# Autodesk Inventor assembly: 165565807 18793263 170831 DFM-12-100-P-A-GF---(fdt_d_0)
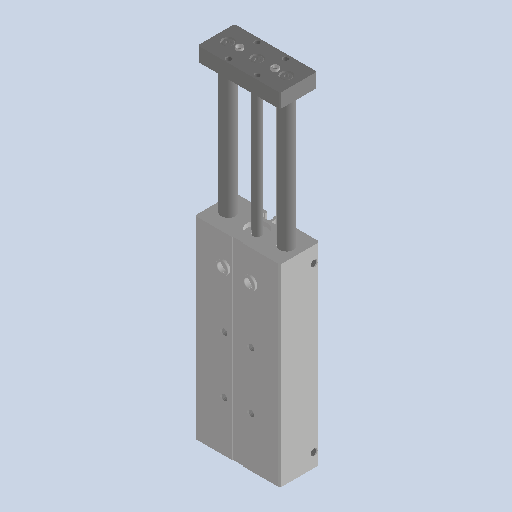
[picture p0: Inventor's stored thumbnail of the model, 512x512]
Saved by Autodesk Inventor 2025.1 (Build 291241000, 241)
## iProperties
Category: PARTsolutions
Created: 2025-06-15
Part Number: 165565807 18793263 170831 DFM-12-100-P-A-GF---(fdt_d_0)
Catalog Web Link: www.cadenas.de
Description: -
Document SubType Name: Assembly
Designer: psAdmin
Mass: 229.263 g
Surface Area: 644.764 cm^2
Volume: 221.571 cm^3
Density: 1.03471 g/cm^3
CREATOR: CADENAS GmbH
Author: Cadenas PARTsolutions
## Documents named in this file (5)
- C:\Users\Erik\Erik\Hochschule\3. Semester\CAD\CAD-Paspa\Useless Box\Kaufteile\Festo_Fuehrungszylinder_100\165565807 18793263 170831 DFM-12-100-P-A-GF---(fdt_d_0).iam
- C:\Users\Erik\Erik\Hochschule\3. Semester\CAD\CAD-Paspa\Useless Box\Kaufteile\Festo_Fuehrungszylinder_100\170831 DFM-12-100-P-A-GF---(Z).ipt
- C:\Users\Erik\Erik\Hochschule\3. Semester\CAD\CAD-Paspa\Useless Box\Kaufteile\Festo_Fuehrungszylinder_100\170831 DFM-12-100-P-A-GF---(K).ipt
- C:\Users\Erik\Erik\Hochschule\3. Semester\CAD\CAD-Paspa\Useless Box\Kaufteile\Festo_Fuehrungszylinder_100\8146543 ZBH-5-B.ipt
- C:\Users\Erik\Erik\Hochschule\3. Semester\CAD\CAD-Paspa\Useless Box\Kaufteile\Festo_Fuehrungszylinder_100\8137184 ZBH-9-B.ipt
## Components (8 placed, 4 different names)
1. 170831 DFM-12-100-P-A-GF---(Z):1 — dfm_z_XY@1 <-> dfm_k_XY@2, dfm_z_Z@1 <-> dfm_k_Z@2, dfm_z_YZ@1 <-> dfm_k_YZ@2, HUELSE2_1_XY@1 <-> insert_XY@5, HUELSE2_1_Z@1 <-> insert_Z@5, HUELSE2_1_YZ@1 <-> insert_YZ@5, HUELSE2_2_XY@1 <-> insert_XY@6, HUELSE2_2_Z@1 <-> insert_Z@6, HUELSE2_2_YZ@1 <-> insert_YZ@6, HUELSE1_1_XY@1 <-> insert_XY@7, HUELSE1_1_Z@1 <-> insert_Z@7, HUELSE1_1_YZ@1 <-> insert_YZ@7, HUELSE1_2_XY@1 <-> insert_XY@8, HUELSE1_2_Z@1 <-> insert_Z@8, HUELSE1_2_YZ@1 <-> insert_YZ@8
2. 170831 DFM-12-100-P-A-GF---(K):1 — dfm_z_XY@1 <-> dfm_k_XY@2, dfm_z_Z@1 <-> dfm_k_Z@2, dfm_z_YZ@1 <-> dfm_k_YZ@2, HUELSE3_1_XY@2 <-> insert_XY@3, HUELSE3_1_Z@2 <-> insert_Z@3, HUELSE3_1_YZ@2 <-> insert_YZ@3, HUELSE3_2_XY@2 <-> insert_XY@4, HUELSE3_2_Z@2 <-> insert_Z@4, HUELSE3_2_YZ@2 <-> insert_YZ@4
3. 8146543 ZBH-5-B:1 — HUELSE3_1_XY@2 <-> insert_XY@3, HUELSE3_1_Z@2 <-> insert_Z@3, HUELSE3_1_YZ@2 <-> insert_YZ@3
4. 8146543 ZBH-5-B:2 — HUELSE3_2_XY@2 <-> insert_XY@4, HUELSE3_2_Z@2 <-> insert_Z@4, HUELSE3_2_YZ@2 <-> insert_YZ@4
5. 8137184 ZBH-9-B:1 — HUELSE2_1_XY@1 <-> insert_XY@5, HUELSE2_1_Z@1 <-> insert_Z@5, HUELSE2_1_YZ@1 <-> insert_YZ@5
6. 8137184 ZBH-9-B:2 — HUELSE2_2_XY@1 <-> insert_XY@6, HUELSE2_2_Z@1 <-> insert_Z@6, HUELSE2_2_YZ@1 <-> insert_YZ@6
7. 8146543 ZBH-5-B:3 — HUELSE1_1_XY@1 <-> insert_XY@7, HUELSE1_1_Z@1 <-> insert_Z@7, HUELSE1_1_YZ@1 <-> insert_YZ@7
8. 8146543 ZBH-5-B:4 — HUELSE1_2_XY@1 <-> insert_XY@8, HUELSE1_2_Z@1 <-> insert_Z@8, HUELSE1_2_YZ@1 <-> insert_YZ@8
## Relationships (21: Mate 12, Angle 7, Flush 2)
- dfm_z_XY@1 <-> dfm_k_XY@2 [Mate]: 170831 DFM-12-100-P-A-GF---(Z):1 ↔ 170831 DFM-12-100-P-A-GF---(K):1
- dfm_z_Z@1 <-> dfm_k_Z@2 [Mate]: 170831 DFM-12-100-P-A-GF---(Z):1 ↔ 170831 DFM-12-100-P-A-GF---(K):1
- dfm_z_YZ@1 <-> dfm_k_YZ@2 [Angle] (0 deg): 170831 DFM-12-100-P-A-GF---(Z):1 ↔ 170831 DFM-12-100-P-A-GF---(K):1
- HUELSE3_1_XY@2 <-> insert_XY@3 [Flush]: 170831 DFM-12-100-P-A-GF---(K):1 ↔ 8146543 ZBH-5-B:1
- HUELSE3_1_Z@2 <-> insert_Z@3 [Mate]: 170831 DFM-12-100-P-A-GF---(K):1 ↔ 8146543 ZBH-5-B:1
- HUELSE3_1_YZ@2 <-> insert_YZ@3 [Angle] (0 deg): 170831 DFM-12-100-P-A-GF---(K):1 ↔ 8146543 ZBH-5-B:1
- HUELSE3_2_XY@2 <-> insert_XY@4 [Flush]: 170831 DFM-12-100-P-A-GF---(K):1 ↔ 8146543 ZBH-5-B:2
- HUELSE3_2_Z@2 <-> insert_Z@4 [Mate]: 170831 DFM-12-100-P-A-GF---(K):1 ↔ 8146543 ZBH-5-B:2
- HUELSE3_2_YZ@2 <-> insert_YZ@4 [Angle] (0 deg): 170831 DFM-12-100-P-A-GF---(K):1 ↔ 8146543 ZBH-5-B:2
- HUELSE2_1_XY@1 <-> insert_XY@5 [Mate]: 170831 DFM-12-100-P-A-GF---(Z):1 ↔ 8137184 ZBH-9-B:1
- HUELSE2_1_Z@1 <-> insert_Z@5 [Mate]: 170831 DFM-12-100-P-A-GF---(Z):1 ↔ 8137184 ZBH-9-B:1
- HUELSE2_1_YZ@1 <-> insert_YZ@5 [Angle] (0 deg): 170831 DFM-12-100-P-A-GF---(Z):1 ↔ 8137184 ZBH-9-B:1
- HUELSE2_2_XY@1 <-> insert_XY@6 [Mate]: 170831 DFM-12-100-P-A-GF---(Z):1 ↔ 8137184 ZBH-9-B:2
- HUELSE2_2_Z@1 <-> insert_Z@6 [Mate]: 170831 DFM-12-100-P-A-GF---(Z):1 ↔ 8137184 ZBH-9-B:2
- HUELSE2_2_YZ@1 <-> insert_YZ@6 [Angle] (0 deg): 170831 DFM-12-100-P-A-GF---(Z):1 ↔ 8137184 ZBH-9-B:2
- HUELSE1_1_XY@1 <-> insert_XY@7 [Mate]: 170831 DFM-12-100-P-A-GF---(Z):1 ↔ 8146543 ZBH-5-B:3
- HUELSE1_1_Z@1 <-> insert_Z@7 [Mate]: 170831 DFM-12-100-P-A-GF---(Z):1 ↔ 8146543 ZBH-5-B:3
- HUELSE1_1_YZ@1 <-> insert_YZ@7 [Angle] (0 deg): 170831 DFM-12-100-P-A-GF---(Z):1 ↔ 8146543 ZBH-5-B:3
- HUELSE1_2_XY@1 <-> insert_XY@8 [Mate]: 170831 DFM-12-100-P-A-GF---(Z):1 ↔ 8146543 ZBH-5-B:4
- HUELSE1_2_Z@1 <-> insert_Z@8 [Mate]: 170831 DFM-12-100-P-A-GF---(Z):1 ↔ 8146543 ZBH-5-B:4
- HUELSE1_2_YZ@1 <-> insert_YZ@8 [Angle] (0 deg): 170831 DFM-12-100-P-A-GF---(Z):1 ↔ 8146543 ZBH-5-B:4
